# Autodesk Inventor assembly: Schalter
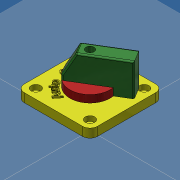
[picture p0: Inventor's stored thumbnail of the model, 180x180]
Saved by Autodesk Inventor 2019 (Build 230136000, 136)
## iProperties
Created: 2020-08-07
Part Number: Schalter
Material: Generisch
Document SubType Name: Assembly
Designer: Stefan
Mass: 23.414 g
Surface Area: 124.122 cm^2
Volume: 23.414 cm^3
Density: 1 g/cm^3
Author: Stefan
## Documents named in this file (4)
- C:\Users\User\OneDrive\Dokumente\Inventor\Absauganlage\Schalter.iam
- C:\Users\User\OneDrive\Dokumente\Inventor\Absauganlage\Schalter_Platte_Auto-Manuell.ipt
- C:\Users\User\OneDrive\Dokumente\Inventor\Absauganlage\Schalter_Basis.ipt
- C:\Users\User\OneDrive\Dokumente\Inventor\Absauganlage\Schalter_Knauf.ipt
## Components (3 placed, 3 different names)
1. Schalter_Platte_Auto-Manuell:1 — Passend:4, Passend:5
2. Schalter_Basis:1 — Passend:1, Passend:2, Passend:3, Passend:4, Passend:5
3. Schalter_Knauf:1 — Passend:1, Passend:2, Passend:3
## Relationships (5: Mate 5)
- Passend:1 [Mate]: Schalter_Basis:1 ↔ Schalter_Knauf:1
- Passend:2 [Mate]: Schalter_Basis:1 ↔ Schalter_Knauf:1
- Passend:3 [Mate]: Schalter_Basis:1 ↔ Schalter_Knauf:1
- Passend:4 [Mate]: Schalter_Platte_Auto-Manuell:1 ↔ Schalter_Basis:1
- Passend:5 [Mate] (1 mm): Schalter_Platte_Auto-Manuell:1 ↔ Schalter_Basis:1
